# Autodesk Inventor assembly: sub_assy_robot_arm_link1
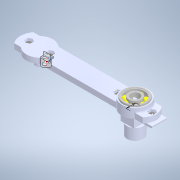
[picture p0: Inventor's stored thumbnail of the model, 180x180]
Saved by Autodesk Inventor 2021 (Build 250183000, 183)
## iProperties
Created: 2021-01-13
Part Number: sub_assy_robot_arm_link1
Document SubType Name: Assembly
Designer: Sam
Sending System: SolidWorks 2020
Last Author: Ben
Last Saved: 2021-01-14
Author: Sam
## Documents named in this file (9)
- D:\OneDrive\MSc Robotics\GIC\RobotKinematics-Remote\3D CAD\Autodesk\23022021\sub_assy_robot_arm_link1.iam
- D:\OneDrive\MSc Robotics\GIC\RobotKinematics-Remote\3D CAD\Autodesk\23022021\robot_arm_link_bearing_insert_mk1.ipt
- D:\OneDrive\MSc Robotics\GIC\RobotKinematics-Remote\3D CAD\Autodesk\23022021\Df_Robot_stepper_FIT0503.ipt
- D:\OneDrive\MSc Robotics\GIC\RobotKinematics-Remote\3D CAD\Autodesk\23022021\608_Z.iam
- D:\OneDrive\MSc Robotics\GIC\RobotKinematics-Remote\3D CAD\Autodesk\23022021\DfRobot_stepper_FIT0503_mount_v4.ipt
- D:\OneDrive\MSc Robotics\GIC\RobotKinematics-Remote\3D CAD\Autodesk\23022021\arm_1_v2.ipt
- C:\Users\Sam\Documents\Inventor\Content Center Files\R2021\en-US\BS 4183(2)\BS 4183 - M3 x 6(1) I.ipt
- C:\Users\Sam\Documents\Inventor\Content Center Files\R2021\en-US\BS 4183(1)\BS 4183 - M3(1).ipt
- C:\Users\Sam\Documents\Inventor\Content Center Files\R2021\en-US\BS 4183(6)\BS 4183 - M3 x 6(2) II.ipt
## Components (15 placed, 8 different names)
1. arm_1_v2:1 — Mate:1, Mate:2, Mate:3, Mate:4, Mate:5, Mate:6, Mate:7, Mate:16, Mate:18, Mate:20, Mate:21, Mate:22, Mate:23, Mate:24
2. robot_arm_link_bearing_insert_mk1:1 — Mate:1, Mate:2, Mate:3
3. DfRobot_stepper_FIT0503_mount_v4:1 — Mate:6, Mate:7, Mate:8, Mate:9, Mate:10, Mate:11, Mate:12, Mate:13, Mate:14, Mate:15, Mate:17, Mate:19
4. Df_Robot_stepper_FIT0503:1 — Mate:9, Mate:10, Mate:11
5. 608_Z:1 [sub-assembly] — Mate:4, Mate:5
6. BS 4183 Cross Recessed Flat Countersunk Head Machine Screw - Metric M3 x 6:1 — Mate:12
7. BS 4183 - Metric M3:1 — Mate:15, Mate:16
8. BS 4183 Cross Recessed Flat Countersunk Head Machine Screw - Metric M3 x 6:2 — Mate:13
9. BS 4183 Cross Recessed Flat Countersunk Head Machine Screw - Metric M3 x 6:3 — Mate:14
10. BS 4183 - Metric M3:2 — Mate:17, Mate:18
11. BS 4183 - Metric M3:3 — Mate:19, Mate:20
12. BS 4183 Slotted Flat Countersunk Head Machine Screw - Metric M3 x 6:1
13. BS 4183 - Metric M3:4 — Mate:21, Mate:22
14. BS 4183 Slotted Flat Countersunk Head Machine Screw - Metric M3 x 6:2
15. BS 4183 - Metric M3:5 — Mate:23, Mate:24
## Relationships (24: Mate 24)
- Mate:1: arm_1_v2:1 ↔ robot_arm_link_bearing_insert_mk1:1
- Mate:2: arm_1_v2:1 ↔ robot_arm_link_bearing_insert_mk1:1
- Mate:3: arm_1_v2:1 ↔ robot_arm_link_bearing_insert_mk1:1
- Mate:4: arm_1_v2:1 ↔ 608_Z:1
- Mate:5: arm_1_v2:1 ↔ 608_Z:1
- Mate:6: arm_1_v2:1 ↔ DfRobot_stepper_FIT0503_mount_v4:1
- Mate:7: arm_1_v2:1 ↔ DfRobot_stepper_FIT0503_mount_v4:1
- Mate:8: DfRobot_stepper_FIT0503_mount_v4:1
- Mate:9: DfRobot_stepper_FIT0503_mount_v4:1 ↔ Df_Robot_stepper_FIT0503:1
- Mate:10: DfRobot_stepper_FIT0503_mount_v4:1 ↔ Df_Robot_stepper_FIT0503:1
- Mate:11: DfRobot_stepper_FIT0503_mount_v4:1 ↔ Df_Robot_stepper_FIT0503:1
- Mate:12: DfRobot_stepper_FIT0503_mount_v4:1 ↔ BS 4183 Cross Recessed Flat Countersunk Head Machine Screw - Metric M3 x 6:1
- Mate:13: DfRobot_stepper_FIT0503_mount_v4:1 ↔ BS 4183 Cross Recessed Flat Countersunk Head Machine Screw - Metric M3 x 6:2
- Mate:14: DfRobot_stepper_FIT0503_mount_v4:1 ↔ BS 4183 Cross Recessed Flat Countersunk Head Machine Screw - Metric M3 x 6:3
- Mate:15: DfRobot_stepper_FIT0503_mount_v4:1 ↔ BS 4183 - Metric M3:1
- Mate:16: arm_1_v2:1 ↔ BS 4183 - Metric M3:1
- Mate:17: DfRobot_stepper_FIT0503_mount_v4:1 ↔ BS 4183 - Metric M3:2
- Mate:18: arm_1_v2:1 ↔ BS 4183 - Metric M3:2
- Mate:19: DfRobot_stepper_FIT0503_mount_v4:1 ↔ BS 4183 - Metric M3:3
- Mate:20: arm_1_v2:1 ↔ BS 4183 - Metric M3:3
- Mate:21: arm_1_v2:1 ↔ BS 4183 - Metric M3:4
- Mate:22: arm_1_v2:1 ↔ BS 4183 - Metric M3:4
- Mate:23: arm_1_v2:1 ↔ BS 4183 - Metric M3:5
- Mate:24: arm_1_v2:1 ↔ BS 4183 - Metric M3:5
